# Autodesk Inventor assembly: Assembly2
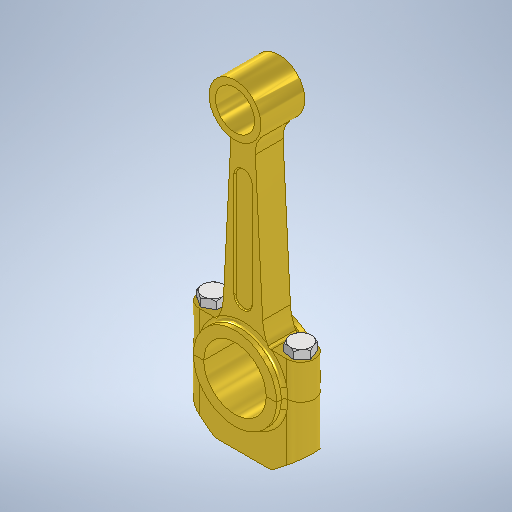
[picture p0: Inventor's stored thumbnail of the model, 512x512]
Saved by Autodesk Inventor 2025.2 (Build 292293000, 293)
## iProperties
Created: 2025-07-02
Part Number: Assembly2
Document SubType Name: Assembly
Designer: akmal
Author: akmal
## Documents named in this file (5)
- C:\Users\akmal\OneDrive\Desktop\Akmal\Work\Assembly2.iam
- C:\Users\akmal\OneDrive\Desktop\Akmal\Work\Connection Road Head.ipt
- C:\Users\akmal\OneDrive\Desktop\Akmal\Work\Part3.ipt
- C:\Users\akmal\OneDrive\Desktop\Akmal\Work\M10 Bolt.ipt
- C:\Users\akmal\OneDrive\Desktop\Akmal\Work\M10 Nut.ipt
## Components (6 placed, 4 different names)
1. Connection Road Head:1 — Mate:1, Mate:2, Mate:3, Mate:4, Mate:11, Mate:12
2. Part3:1 — Mate:1, Mate:2, Mate:3, Mate:4, Mate:5, Mate:6, Mate:7, Mate:8
3. M10 Bolt:1 — Mate:6, Mate:7, Mate:10
4. M10 Bolt:2 — Mate:5, Mate:8, Mate:9
5. M10 Nut:1 — Mate:10, Mate:11
6. M10 Nut:2 — Mate:9, Mate:12
## Relationships (12: Mate 12)
- Mate:1: Connection Road Head:1 ↔ Part3:1
- Mate:2: Connection Road Head:1 ↔ Part3:1
- Mate:3: Connection Road Head:1 ↔ Part3:1
- Mate:4: Connection Road Head:1 ↔ Part3:1
- Mate:5: Part3:1 ↔ M10 Bolt:2
- Mate:6: Part3:1 ↔ M10 Bolt:1
- Mate:7: Part3:1 ↔ M10 Bolt:1
- Mate:8: Part3:1 ↔ M10 Bolt:2
- Mate:9: M10 Bolt:2 ↔ M10 Nut:2
- Mate:10: M10 Bolt:1 ↔ M10 Nut:1
- Mate:11: Connection Road Head:1 ↔ M10 Nut:1
- Mate:12: Connection Road Head:1 ↔ M10 Nut:2
